# Autodesk Inventor assembly: X_Carriage_V2_0
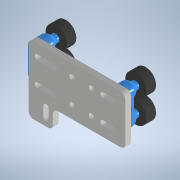
[picture p0: Inventor's stored thumbnail of the model, 180x180]
Saved by Autodesk Inventor 2021 (Build 250183000, 183)
## iProperties
Created: 2021-06-13
Part Number: X_Carriage_V2_0
Document SubType Name: Assembly
Designer: Jorian Brusind
Author: Jorian Brusind
## Documents named in this file (6)
- C:\Users\Jorian Brusind\Documents\GitHub\PersonalProjects\HyperRail\Inventor Files\X_Carriage_V2_0.iam
- C:\Users\Jorian Brusind\Documents\GitHub\PersonalProjects\HyperRail\Inventor Files\X_Carriage_Plate.ipt
- C:\Users\Jorian Brusind\Documents\GitHub\PersonalProjects\HyperRail\Inventor Files\11mm_BearingWheel.ipt
- C:\Users\Jorian Brusind\Documents\GitHub\PersonalProjects\HyperRail\Inventor Files\4mm_Roller_Spacer_simple.ipt
- C:\Users\Jorian Brusind\Documents\GitHub\PersonalProjects\HyperRail\Inventor Files\Rollder_Spacer_Single.ipt
- C:\Users\Jorian Brusind\Documents\GitHub\PersonalProjects\HyperRail\Inventor Files\10mm_Idle_Pulley.ipt
## Components (9 placed, 5 different names)
1. X_Carriage_Plate:1 — Mate:7, Mate:14, Mate:27, Mate:29, Mate:33, Mate:42, Angle:1, Angle:2, Mate:45
2. 11mm_BearingWheel:1 — Flush:2, Mate:43
3. 11mm_BearingWheel:4 — Flush:2, Mate:7, Mate:44
4. 4mm_Roller_Spacer_simple:2 — Mate:14, Mate:42, Angle:1, Mate:46, Mate:47, Mate:48
5. Rollder_Spacer_Single:1 — Mate:27, Mate:28, Mate:29, Mate:30
6. 10mm_Idle_Pulley:1 — Mate:28, Mate:30
7. 4mm_Roller_Spacer_simple:3 — Mate:33, Mate:43, Mate:44, Angle:2, Mate:45
8. 11mm_BearingWheel:5 — Mate:46, Flush:3, Mate:48
9. 11mm_BearingWheel:6 — Mate:47, Flush:3
## Relationships (18: Mate 14, Flush 2, Angle 2)
- Flush:2: 11mm_BearingWheel:1 ↔ 11mm_BearingWheel:4
- Mate:7 (20 mm): X_Carriage_Plate:1 ↔ 11mm_BearingWheel:4
- Mate:14: X_Carriage_Plate:1 ↔ 4mm_Roller_Spacer_simple:2
- Mate:27: X_Carriage_Plate:1 ↔ Rollder_Spacer_Single:1
- Mate:28: Rollder_Spacer_Single:1 ↔ 10mm_Idle_Pulley:1
- Mate:29: X_Carriage_Plate:1 ↔ Rollder_Spacer_Single:1
- Mate:30: Rollder_Spacer_Single:1 ↔ 10mm_Idle_Pulley:1
- Mate:33: X_Carriage_Plate:1 ↔ 4mm_Roller_Spacer_simple:3
- Mate:42 (-12.5 mm): X_Carriage_Plate:1 ↔ 4mm_Roller_Spacer_simple:2
- Angle:1 (0 deg): X_Carriage_Plate:1 ↔ 4mm_Roller_Spacer_simple:2
- Mate:43: 11mm_BearingWheel:1 ↔ 4mm_Roller_Spacer_simple:3
- Mate:44: 11mm_BearingWheel:4 ↔ 4mm_Roller_Spacer_simple:3
- Angle:2 (0 deg): X_Carriage_Plate:1 ↔ 4mm_Roller_Spacer_simple:3
- Mate:45 (-12.5 mm): X_Carriage_Plate:1 ↔ 4mm_Roller_Spacer_simple:3
- Mate:46: 4mm_Roller_Spacer_simple:2 ↔ 11mm_BearingWheel:5
- Mate:47: 4mm_Roller_Spacer_simple:2 ↔ 11mm_BearingWheel:6
- Flush:3: 11mm_BearingWheel:5 ↔ 11mm_BearingWheel:6
- Mate:48: 4mm_Roller_Spacer_simple:2 ↔ 11mm_BearingWheel:5
